# Autodesk Inventor assembly: ASY SLM 1610 charging hatch
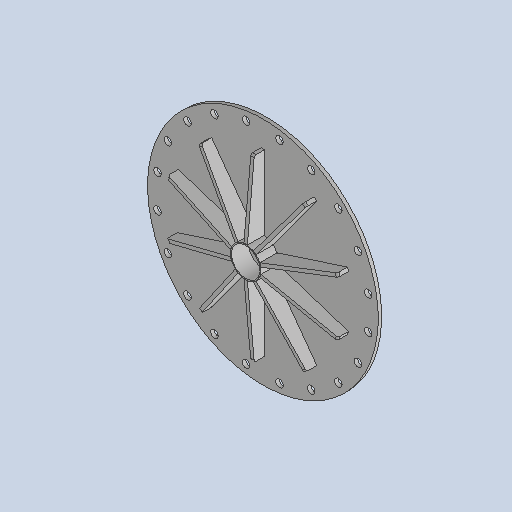
[picture p0: Inventor's stored thumbnail of the model, 512x512]
Saved by Autodesk Inventor 2025.4 (Build 294407000, 407)
## iProperties
Created: 2025-04-22
Part Number: ASY SLM 1610 charging hatch
Document SubType Name: Assembly
Designer: user
Mass: 9483.1 g
Surface Area: 9977.57 cm^2
Volume: 3616.18 cm^3
Density: 2.6224 g/cm^3
Author: user
## Documents named in this file (4)
- C:\Users\admin\Documents\Inventor\NDA-Nyyda\ASY PNS 1610 charging hatch.iam
- C:\Users\admin\Documents\Inventor\NDA-Nyyda\SLM 1621 charging hatch D940.ipt
- C:\Users\admin\Documents\Inventor\NDA-Nyyda\SLM 1614 charging hatch reinf 500mm.ipt
- C:\Users\admin\Documents\Inventor\NDA-Nyyda\SLM 1611 hatch tube 500mm.ipt
## Components (12 placed, 3 different names)
1. PNS 1621 charging hatch D1000.ipt:1 — Rigid:1, Flush:1
2. PNS 1711 hatch tube 500mm.ipt:1 — Rigid:1
3. PNS 1614 charging hatch reinf 500mm.ipt:1 — Mate:1, Flush:1, Mate:2, Mate:3
4. PNS 1614 charging hatch reinf 500mm.ipt:2
5. PNS 1614 charging hatch reinf 500mm.ipt:3
6. PNS 1614 charging hatch reinf 500mm.ipt:4
7. PNS 1614 charging hatch reinf 500mm.ipt:5
8. PNS 1614 charging hatch reinf 500mm.ipt:6
9. PNS 1614 charging hatch reinf 500mm.ipt:7
10. PNS 1614 charging hatch reinf 500mm.ipt:8
11. PNS 1614 charging hatch reinf 500mm.ipt:9
12. PNS 1614 charging hatch reinf 500mm.ipt:10
## Component patterns: (10 elements, first: PNS 1614 charging hatch reinf 500mm.ipt:1)
## Relationships (5: Mate 3, WeldJoint 1, Flush 1)
- Rigid:1 [WeldJoint]: PNS 1621 charging hatch D1000.ipt:1 ↔ PNS 1711 hatch tube 500mm.ipt:1
- Mate:1: PNS 1614 charging hatch reinf 500mm.ipt:1
- Flush:1: PNS 1621 charging hatch D1000.ipt:1 ↔ PNS 1614 charging hatch reinf 500mm.ipt:1
- Mate:2: PNS 1614 charging hatch reinf 500mm.ipt:1
- Mate:3: PNS 1614 charging hatch reinf 500mm.ipt:1
